# Autodesk Inventor assembly: assembly
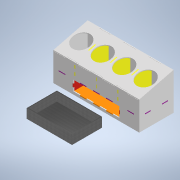
[picture p0: Inventor's stored thumbnail of the model, 180x180]
Saved by Autodesk Inventor 2020 (Build 240168000, 168)
## iProperties
Created: 2020-02-22
Part Number: assembly
Document SubType Name: Assembly
Designer: udvarhelyi
Author: udvarhelyi
## Documents named in this file (13)
- C:\Users\udvarhelyi\Desktop\Escape_4maisons\assembly.iam
- C:\Users\udvarhelyi\Desktop\Escape_4maisons\back.ipt
- C:\Users\udvarhelyi\Desktop\Escape_4maisons\base.ipt
- C:\Users\udvarhelyi\Desktop\Escape_4maisons\front.ipt
- C:\Users\udvarhelyi\Desktop\Escape_4maisons\side.ipt
- C:\Users\udvarhelyi\Desktop\Escape_4maisons\top.ipt
- C:\Users\udvarhelyi\Desktop\Escape_4maisons\in_separator.ipt
- C:\Users\udvarhelyi\Desktop\Escape_4maisons\base_shelf.ipt
- C:\Users\udvarhelyi\Desktop\Escape_4maisons\side_shelf.ipt
- C:\Users\udvarhelyi\Desktop\Escape_4maisons\shelf_bottom.ipt
- C:\Users\udvarhelyi\Desktop\Escape_4maisons\shelf_left_right.ipt
- C:\Users\udvarhelyi\Desktop\Escape_4maisons\shelf_front_back.ipt
- C:\Users\udvarhelyi\Desktop\Escape_4maisons\glass_separator.ipt
## Components (18 placed, 12 different names)
1. back:1 — Mate:1, Flush:1, Mate:6, Flush:9, Flush:19, Mate:21, Mate:22, Flush:20, Mate:23, Mate:24, Flush:21, Mate:25, Mate:26
2. base:1 — Mate:1, Flush:1, Mate:6, Flush:6, Flush:8, Flush:10, Flush:12, Flush:13, Flush:15, Mate:9
3. side:1 — Flush:6, Flush:14, Flush:15, Flush:16, Flush:17, Mate:8, Flush:18, Mate:10, Mate:11
4. side:2 — Flush:8, Flush:9, Flush:11, Flush:12
5. front:1 — Flush:10, Flush:11, Flush:13, Flush:14, Mate:7, Flush:32, Mate:34, Mate:35, Flush:34, Mate:36, Mate:37, Flush:35, Mate:38, Mate:39
6. top:1 — Flush:16, Flush:17, Mate:7, Mate:8
7. in_separator:1 — Flush:18, Mate:10, Mate:11, Flush:33
8. base_shelf:1 — Flush:19, Mate:21, Mate:22, Mate:33
9. side_shelf:1 — Flush:21, Mate:25, Mate:26, Mate:32
10. side_shelf:2 — Flush:20, Mate:23, Mate:24
11. shelf_bottom:1 — Flush:24, Flush:25, Mate:28, Flush:30, Mate:33
12. shelf_left_right:1 — Flush:24, Flush:25, Mate:28, Flush:26, Flush:27, Mate:29, Flush:28, Flush:29, Mate:30
13. shelf_front_back:1 — Flush:26, Flush:27, Mate:29
14. shelf_front_back:2 — Flush:28, Flush:29, Mate:30, Flush:31, Mate:31
15. shelf_left_right:2 — Flush:30, Flush:31, Mate:31, Mate:32
16. glass_separator:1 — Flush:32, Mate:34, Mate:35, Flush:33
17. glass_separator:2 — Flush:34, Mate:36, Mate:37
18. glass_separator:3 — Flush:35, Mate:38, Mate:39
## Relationships (53: Flush 28, Mate 25)
- Mate:1: back:1 ↔ base:1
- Flush:1: back:1 ↔ base:1
- Mate:6: back:1 ↔ base:1
- Flush:6: base:1 ↔ side:1
- Flush:8: base:1 ↔ side:2
- Flush:9: back:1 ↔ side:2
- Flush:10: base:1 ↔ front:1
- Flush:11: side:2 ↔ front:1
- Flush:12: base:1 ↔ side:2
- Flush:13: base:1 ↔ front:1
- Flush:14: side:1 ↔ front:1
- Flush:15: base:1 ↔ side:1
- Flush:16: side:1 ↔ top:1
- Flush:17: side:1 ↔ top:1
- Mate:7: front:1 ↔ top:1
- Mate:8: side:1 ↔ top:1
- Mate:9: base:1
- Flush:18: side:1 ↔ in_separator:1
- Mate:10: side:1 ↔ in_separator:1
- Mate:11: side:1 ↔ in_separator:1
- Flush:19: back:1 ↔ base_shelf:1
- Mate:21: back:1 ↔ base_shelf:1
- Mate:22: back:1 ↔ base_shelf:1
- Flush:20: back:1 ↔ side_shelf:2
- Mate:23: back:1 ↔ side_shelf:2
- Mate:24: back:1 ↔ side_shelf:2
- Flush:21: back:1 ↔ side_shelf:1
- Mate:25: back:1 ↔ side_shelf:1
- Mate:26: back:1 ↔ side_shelf:1
- Flush:24: shelf_bottom:1 ↔ shelf_left_right:1
- Flush:25: shelf_bottom:1 ↔ shelf_left_right:1
- Mate:28: shelf_bottom:1 ↔ shelf_left_right:1
- Flush:26: shelf_left_right:1 ↔ shelf_front_back:1
- Flush:27: shelf_left_right:1 ↔ shelf_front_back:1
- Mate:29: shelf_left_right:1 ↔ shelf_front_back:1
- Flush:28: shelf_left_right:1 ↔ shelf_front_back:2
- Flush:29: shelf_left_right:1 ↔ shelf_front_back:2
- Mate:30: shelf_left_right:1 ↔ shelf_front_back:2
- Flush:30: shelf_bottom:1 ↔ shelf_left_right:2
- Flush:31: shelf_front_back:2 ↔ shelf_left_right:2
- Mate:31: shelf_front_back:2 ↔ shelf_left_right:2
- Mate:32: side_shelf:1 ↔ shelf_left_right:2
- Mate:33: base_shelf:1 ↔ shelf_bottom:1
- Flush:32: front:1 ↔ glass_separator:1
- Mate:34: front:1 ↔ glass_separator:1
- Mate:35: front:1 ↔ glass_separator:1
- Flush:33: in_separator:1 ↔ glass_separator:1
- Flush:34: front:1 ↔ glass_separator:2
- Mate:36: front:1 ↔ glass_separator:2
- Mate:37: front:1 ↔ glass_separator:2
- Flush:35: front:1 ↔ glass_separator:3
- Mate:38: front:1 ↔ glass_separator:3
- Mate:39: front:1 ↔ glass_separator:3
